# Autodesk Inventor assembly: Nema 17
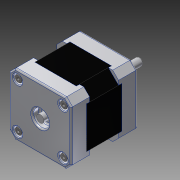
[picture p0: Inventor's stored thumbnail of the model, 180x180]
Saved by Autodesk Inventor 2016 (Build 200138000, 138)
## iProperties
Created: 2015-09-21
Part Number: Nema 17
Document SubType Name: Assembly
Designer: Dr Kreigar
Author: Dr Kreigar
## Documents named in this file (6)
- C:\Users\Owner\Documents\REZ_RAP\Nema 17.iam
- C:\Users\Owner\Documents\REZ_RAP\Nema 17 Base.ipt
- C:\Users\Owner\Documents\REZ_RAP\Nema 17 Body.ipt
- C:\Users\Owner\Documents\REZ_RAP\Nema 17 Top.ipt
- C:\Users\Owner\Documents\REZ_RAP\Nema 17 Shaft.ipt
- C:\Users\Owner\Documents\REZ_RAP\ISO 4762 - M2.5 x 6DIN EN ISO.ipt
## Components (8 placed, 5 different names)
1. Nema 17 Base:1 — Flush:1, Flush:3, Insert:1, Insert:2, Insert:3, Insert:4
2. Nema 17 Body:1 — Flush:1, Mate:1, Mate:2, Flush:2
3. Nema 17 Top:1 — Mate:1, Mate:2, Flush:2, Mate:3
4. Nema 17 Shaft:1 — Mate:3, Flush:3
5. DIN EN ISO 4762 M2.5 x 6:1 — Insert:1
6. DIN EN ISO 4762 M2.5 x 6:2 — Insert:2
7. DIN EN ISO 4762 M2.5 x 6:3 — Insert:3
8. DIN EN ISO 4762 M2.5 x 6:4 — Insert:4
## Relationships (10: Insert 4, Flush 3, Mate 3)
- Flush:1: Nema 17 Base:1 ↔ Nema 17 Body:1
- Mate:1: Nema 17 Body:1 ↔ Nema 17 Top:1
- Mate:2: Nema 17 Body:1 ↔ Nema 17 Top:1
- Flush:2: Nema 17 Body:1 ↔ Nema 17 Top:1
- Mate:3: Nema 17 Top:1 ↔ Nema 17 Shaft:1
- Flush:3: Nema 17 Base:1 ↔ Nema 17 Shaft:1
- Insert:1: Nema 17 Base:1 ↔ DIN EN ISO 4762 M2.5 x 6:1
- Insert:2: Nema 17 Base:1 ↔ DIN EN ISO 4762 M2.5 x 6:2
- Insert:3: Nema 17 Base:1 ↔ DIN EN ISO 4762 M2.5 x 6:3
- Insert:4: Nema 17 Base:1 ↔ DIN EN ISO 4762 M2.5 x 6:4
